# Autodesk Inventor assembly: hph_002
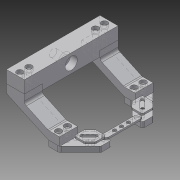
[picture p0: Inventor's stored thumbnail of the model, 180x180]
Saved by Autodesk Inventor 2014 (Build 180170000, 170)
## iProperties
Created: 2014-03-27
Part Number: hph_002
Document SubType Name: Assembly
Designer: stephenholtz
Author: stephenholtz
## Documents named in this file (7)
- C:\Users\stephenholtz\Dropbox\grad_school_docs\sabatini_lab_rotation\headpost_design\hph_001.iam
- C:\Users\stephenholtz\Dropbox\grad_school_docs\sabatini_lab_rotation\headpost_design\hph_C_001.ipt
- C:\Users\stephenholtz\Dropbox\grad_school_docs\sabatini_lab_rotation\headpost_design\hph_B_001.ipt
- C:\Users\stephenholtz\Dropbox\grad_school_docs\sabatini_lab_rotation\headpost_design\hph_A_001_left.ipt
- C:\Users\stephenholtz\Dropbox\grad_school_docs\sabatini_lab_rotation\headpost_design\hph_A_001_right.ipt
- C:\Users\stephenholtz\Dropbox\grad_school_docs\sabatini_lab_rotation\headpost_design\hph_D_001.ipt
- C:\Users\stephenholtz\Dropbox\grad_school_docs\sabatini_lab_rotation\headpost_design\hp_thick_001.ipt
## Components (8 placed, 6 different names)
1. hph_C_001:1 — Mate:1, Mate:2, Mate:5, Mate:6, Mate:7, Mate:8
2. hph_B_001:1 — Mate:1, Mate:3, Mate:5, Mate:6, Mate:9, Mate:10
3. hph_B_001:2 — Mate:2, Mate:4, Mate:7, Mate:8, Mate:11, Mate:12
4. hph_A_001_left:1 — Mate:4, Mate:11, Mate:12, Mate:13, Mate:15, Tangent:3, Tangent:4
5. hph_A_001_right:1 — Mate:3, Mate:9, Mate:10, Mate:14, Mate:16, Tangent:1, Tangent:2
6. hph_D_001:1 — Mate:14, Tangent:1, Tangent:2
7. hph_D_001:2 — Mate:13, Tangent:3, Tangent:4
8. hp_thick_001:1 — Mate:15, Mate:16
## Relationships (20: Mate 16, Tangent 4)
- Mate:1: hph_C_001:1 ↔ hph_B_001:1
- Mate:2: hph_C_001:1 ↔ hph_B_001:2
- Mate:3: hph_B_001:1 ↔ hph_A_001_right:1
- Mate:4: hph_B_001:2 ↔ hph_A_001_left:1
- Mate:5: hph_C_001:1 ↔ hph_B_001:1
- Mate:6: hph_C_001:1 ↔ hph_B_001:1
- Mate:7: hph_C_001:1 ↔ hph_B_001:2
- Mate:8: hph_C_001:1 ↔ hph_B_001:2
- Mate:9: hph_B_001:1 ↔ hph_A_001_right:1
- Mate:10: hph_B_001:1 ↔ hph_A_001_right:1
- Mate:11: hph_B_001:2 ↔ hph_A_001_left:1
- Mate:12: hph_B_001:2 ↔ hph_A_001_left:1
- Mate:13 (1.905 mm): hph_A_001_left:1 ↔ hph_D_001:2
- Mate:14 (1.905 mm): hph_A_001_right:1 ↔ hph_D_001:1
- Mate:15 (0.889 mm): hph_A_001_left:1 ↔ hp_thick_001:1
- Mate:16: hph_A_001_right:1 ↔ hp_thick_001:1
- Tangent:1 (0.508 mm): hph_A_001_right:1 ↔ hph_D_001:1
- Tangent:2 (0.508 mm): hph_A_001_right:1 ↔ hph_D_001:1
- Tangent:3 (0.508 mm): hph_A_001_left:1 ↔ hph_D_001:2
- Tangent:4 (0.508 mm): hph_A_001_left:1 ↔ hph_D_001:2
